# Autodesk Inventor assembly: Battery Basket
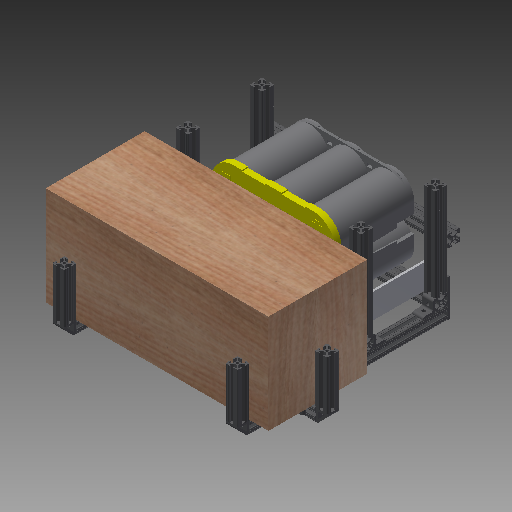
[picture p0: Inventor's stored thumbnail of the model, 512x512]
Saved by Autodesk Inventor 2017 SP1 (Build 210196100, 196)
## iProperties
Created: 2016-04-02
Part Number: Battery Basket
Document SubType Name: Assembly
Designer: hwasserb
Author: hwasserb
## Documents named in this file (14)
- C:\Users\Haden\Desktop\Charlie-CAD-Model\Robot Model\Battery Basket\Battery Basket.iam
- C:\Users\Haden\Desktop\Charlie-CAD-Model\Robot Model\Battery Basket\Back.ipt
- C:\Users\Haden\Desktop\Charlie-CAD-Model\Robot Model\Battery Basket\Bottom.ipt
- C:\Users\Haden\Desktop\Charlie-CAD-Model\Robot Model\Battery Basket\Right Angle.ipt
- C:\Users\Haden\Desktop\Charlie-CAD-Model\Robot Model\Battery Basket\Small Vertical.ipt
- C:\Users\Haden\Desktop\Charlie-CAD-Model\Robot Model\Battery Basket\Optima Battery.ipt
- C:\Users\Haden\Desktop\Charlie-CAD-Model\Robot Model\Battery Basket\Payload Lower Supports.ipt
- C:\Users\Haden\Desktop\Charlie-CAD-Model\Robot Model\Battery Basket\Inside Angle Connector-8020-4119.ipt
- C:\Users\Haden\Desktop\Charlie-CAD-Model\Robot Model\Battery Basket\3 Hole Plate-8020-4118.ipt
- C:\Users\Haden\Desktop\Charlie-CAD-Model\Robot Model\Payload.ipt
- C:\Users\Haden\Desktop\Charlie-CAD-Model\Robot Model\Battery Basket\1.5 Inch Spacer.ipt
- C:\Users\Haden\Desktop\Charlie-CAD-Model\Robot Model\Battery Basket\2 Hole Corner Bracket-8020-4132.ipt
- C:\Users\Haden\Desktop\Charlie-CAD-Model\Robot Model\Battery Basket\Payload Edge Guards.ipt
- C:\Users\Haden\Desktop\Charlie-CAD-Model\Robot Model\Battery Basket\1.75 Inch Spacer.ipt
## Components (39 placed, 13 different names)
1. Back:1 — Mate:23, Flush:3, Flush:4, Mate:64
2. Bottom:1 — Flush:1, Flush:2, Mate:1, Mate:2, Mate:3, Mate:4, Mate:5, Mate:6, Mate:32, Flush:8, Mate:36, Flush:10, Flush:11, Mate:39, Flush:12, Mate:40, Flush:13, Mate:65
3. Bottom:2 — Flush:1, Flush:2, Mate:7, Mate:8, Mate:9, Mate:10, Mate:27, Flush:5, Mate:28, Flush:6, Mate:29, Flush:7, Mate:34, Flush:9, Flush:14, Flush:15, Flush:16
4. Right Angle:1 — Mate:1, Mate:2, Mate:3, Mate:7, Mate:8, Mate:11, Mate:13, Mate:15, Mate:16, Mate:17, Mate:18
5. Right Angle:2 — Mate:4, Mate:5, Mate:6, Mate:9, Mate:10, Mate:12, Mate:14, Mate:19, Mate:20, Mate:21, Mate:22
6. Small Vertical:1 — Mate:13, Mate:15, Mate:16, Mate:26, Mate:47, Flush:27, Flush:28
7. Small Vertical:2 — Mate:14, Mate:19, Mate:20, Mate:45, Flush:21, Flush:22
8. Small Vertical:3 — Mate:12, Mate:21, Mate:22, Mate:44, Flush:23, Flush:24
9. Small Vertical:4 — Mate:11, Mate:17, Mate:18, Mate:23, Flush:3, Flush:4, Mate:46, Flush:25, Flush:26
10. Optima Battery:1 — Mate:26, Mate:64, Mate:65
11. Payload Lower Supports:1 — Mate:27, Flush:5, Mate:30, Mate:31, Mate:37, Flush:14, Mate:41, Flush:17, Insert:6, Flush:34, Flush:37, Mate:51, Mate:54, Flush:38, Mate:59, Flush:41
12. Payload Lower Supports:2 — Mate:28, Flush:6, Mate:33, Mate:35, Mate:38, Flush:13, Mate:42, Flush:18, Mate:43, Flush:19, Flush:20, Insert:5, Flush:35, Mate:50, Flush:36, Mate:57, Flush:39, Mate:58, Flush:40
13. Inside Angle Connector-8020-4119:1 — Mate:29, Flush:7, Mate:30
14. Inside Angle Connector-8020-4119:2 — Mate:33, Mate:34, Flush:9
15. Inside Angle Connector-8020-4119:3 — Mate:31, Mate:32, Flush:8
16. Inside Angle Connector-8020-4119:4 — Mate:35, Mate:36, Flush:10
17. Inside Angle Connector-8020-4119:5 — Mate:37, Flush:11, Mate:39
18. Inside Angle Connector-8020-4119:6 — Mate:38, Flush:12, Mate:40
19. 3 Hole Plate-8020-4118:1 — Mate:41, Flush:16, Flush:17
20. 3 Hole Plate-8020-4118:2 — Mate:42, Flush:15, Flush:18
21. Payload:1 — Mate:43, Flush:19, Flush:20, Flush:45
22. 1.5 Inch Spacer:3 — Mate:46, Flush:25, Flush:26
23. 1.5 Inch Spacer:4 — Mate:44, Flush:23, Flush:24
24. 1.5 Inch Spacer:5 — Mate:47, Flush:27, Flush:28
25. 1.5 Inch Spacer:6 — Mate:45, Flush:21, Flush:22
26. Payload Edge Guards:1 — Insert:4, Flush:43
27. Payload Edge Guards:2 — Insert:2, Flush:44
28. Payload Edge Guards:3 — Flush:34, Insert:7
29. Payload Edge Guards:4 — Flush:35, Insert:8
30. 2 Hole Corner Bracket-8020-4132:1 — Insert:2, Insert:10
31. 2 Hole Corner Bracket-8020-4132:2 — Insert:4, Insert:9
32. 2 Hole Corner Bracket-8020-4132:3 — Insert:5, Insert:8
33. 2 Hole Corner Bracket-8020-4132:4 — Insert:6, Insert:7
34. Inside Angle Connector-8020-4119:7 — Mate:57, Flush:39, Mate:60
35. Inside Angle Connector-8020-4119:8 — Mate:50, Flush:36, Mate:61
36. Inside Angle Connector-8020-4119:9 — Flush:37, Mate:51, Mate:63
37. Inside Angle Connector-8020-4119:10 — Mate:54, Flush:38, Mate:62
38. 1.75 Inch Spacer:1 — Mate:58, Flush:40, Flush:42, Mate:60, Mate:61, Insert:9, Flush:43, Flush:45
39. 1.75 Inch Spacer:2 — Mate:59, Flush:41, Flush:42, Mate:62, Mate:63, Insert:10, Flush:44
## Relationships (105: Mate 57, Flush 40, Insert 8)
- Flush:1: Bottom:1 ↔ Bottom:2
- Flush:2: Bottom:1 ↔ Bottom:2
- Mate:1: Bottom:1 ↔ Right Angle:1
- Mate:2: Bottom:1 ↔ Right Angle:1
- Mate:3: Bottom:1 ↔ Right Angle:1
- Mate:4: Bottom:1 ↔ Right Angle:2
- Mate:5: Bottom:1 ↔ Right Angle:2
- Mate:6: Bottom:1 ↔ Right Angle:2
- Mate:7: Bottom:2 ↔ Right Angle:1
- Mate:8: Bottom:2 ↔ Right Angle:1
- Mate:9: Bottom:2 ↔ Right Angle:2
- Mate:10: Bottom:2 ↔ Right Angle:2
- Mate:11: Right Angle:1 ↔ Small Vertical:4
- Mate:12: Right Angle:2 ↔ Small Vertical:3
- Mate:13: Right Angle:1 ↔ Small Vertical:1
- Mate:14: Right Angle:2 ↔ Small Vertical:2
- Mate:15: Right Angle:1 ↔ Small Vertical:1
- Mate:16: Right Angle:1 ↔ Small Vertical:1
- Mate:17: Right Angle:1 ↔ Small Vertical:4
- Mate:18: Right Angle:1 ↔ Small Vertical:4
- Mate:19: Right Angle:2 ↔ Small Vertical:2
- Mate:20: Right Angle:2 ↔ Small Vertical:2
- Mate:21: Right Angle:2 ↔ Small Vertical:3
- Mate:22: Right Angle:2 ↔ Small Vertical:3
- Mate:23: Back:1 ↔ Small Vertical:4
- Flush:3: Back:1 ↔ Small Vertical:4
- Flush:4 (-76.2 mm): Back:1 ↔ Small Vertical:4
- Mate:26 (38.1 mm): Small Vertical:1 ↔ Optima Battery:1
- Mate:27: Bottom:2 ↔ Payload Lower Supports:1
- Flush:5: Bottom:2 ↔ Payload Lower Supports:1
- Mate:28: Bottom:2 ↔ Payload Lower Supports:2
- Flush:6: Bottom:2 ↔ Payload Lower Supports:2
- Mate:29: Bottom:2 ↔ Inside Angle Connector-8020-4119:1
- Flush:7: Bottom:2 ↔ Inside Angle Connector-8020-4119:1
- Mate:30: Payload Lower Supports:1 ↔ Inside Angle Connector-8020-4119:1
- Mate:31: Payload Lower Supports:1 ↔ Inside Angle Connector-8020-4119:3
- Mate:32: Bottom:1 ↔ Inside Angle Connector-8020-4119:3
- Flush:8: Bottom:1 ↔ Inside Angle Connector-8020-4119:3
- Mate:33: Payload Lower Supports:2 ↔ Inside Angle Connector-8020-4119:2
- Mate:34: Bottom:2 ↔ Inside Angle Connector-8020-4119:2
- Flush:9: Bottom:2 ↔ Inside Angle Connector-8020-4119:2
- Mate:35: Payload Lower Supports:2 ↔ Inside Angle Connector-8020-4119:4
- Mate:36: Bottom:1 ↔ Inside Angle Connector-8020-4119:4
- Flush:10: Bottom:1 ↔ Inside Angle Connector-8020-4119:4
- Mate:37: Payload Lower Supports:1 ↔ Inside Angle Connector-8020-4119:5
- Mate:38: Payload Lower Supports:2 ↔ Inside Angle Connector-8020-4119:6
- Flush:11: Bottom:1 ↔ Inside Angle Connector-8020-4119:5
- Mate:39: Bottom:1 ↔ Inside Angle Connector-8020-4119:5
- Flush:12: Bottom:1 ↔ Inside Angle Connector-8020-4119:6
- Mate:40: Bottom:1 ↔ Inside Angle Connector-8020-4119:6
- Flush:13: Bottom:1 ↔ Payload Lower Supports:2
- Flush:14: Bottom:2 ↔ Payload Lower Supports:1
- Mate:41: Payload Lower Supports:1 ↔ 3 Hole Plate-8020-4118:1
- Mate:42: Payload Lower Supports:2 ↔ 3 Hole Plate-8020-4118:2
- Flush:15: Bottom:2 ↔ 3 Hole Plate-8020-4118:2
- Flush:16: Bottom:2 ↔ 3 Hole Plate-8020-4118:1
- Flush:17: Payload Lower Supports:1 ↔ 3 Hole Plate-8020-4118:1
- Flush:18: Payload Lower Supports:2 ↔ 3 Hole Plate-8020-4118:2
- Mate:43: Payload Lower Supports:2 ↔ Payload:1
- Flush:19: Payload Lower Supports:2 ↔ Payload:1
- Flush:20 (-38.1 mm): Payload Lower Supports:2 ↔ Payload:1
- Mate:44: Small Vertical:3 ↔ 1.5 Inch Spacer:4
- Mate:45: Small Vertical:2 ↔ 1.5 Inch Spacer:6
- Mate:46: Small Vertical:4 ↔ 1.5 Inch Spacer:3
- Mate:47: Small Vertical:1 ↔ 1.5 Inch Spacer:5
- Flush:21: Small Vertical:2 ↔ 1.5 Inch Spacer:6
- Flush:22: Small Vertical:2 ↔ 1.5 Inch Spacer:6
- Flush:23: Small Vertical:3 ↔ 1.5 Inch Spacer:4
- Flush:24: Small Vertical:3 ↔ 1.5 Inch Spacer:4
- Flush:25: Small Vertical:4 ↔ 1.5 Inch Spacer:3
- Flush:26: Small Vertical:4 ↔ 1.5 Inch Spacer:3
- Flush:27: Small Vertical:1 ↔ 1.5 Inch Spacer:5
- Flush:28: Small Vertical:1 ↔ 1.5 Inch Spacer:5
- Insert:2: Payload Edge Guards:2 ↔ 2 Hole Corner Bracket-8020-4132:1
- Insert:4: Payload Edge Guards:1 ↔ 2 Hole Corner Bracket-8020-4132:2
- Insert:5: Payload Lower Supports:2 ↔ 2 Hole Corner Bracket-8020-4132:3
- Insert:6: Payload Lower Supports:1 ↔ 2 Hole Corner Bracket-8020-4132:4
- Flush:34: Payload Lower Supports:1 ↔ Payload Edge Guards:3
- Flush:35: Payload Lower Supports:2 ↔ Payload Edge Guards:4
- Insert:7: Payload Edge Guards:3 ↔ 2 Hole Corner Bracket-8020-4132:4
- Insert:8: Payload Edge Guards:4 ↔ 2 Hole Corner Bracket-8020-4132:3
- Mate:50: Payload Lower Supports:2 ↔ Inside Angle Connector-8020-4119:8
- Flush:36: Payload Lower Supports:2 ↔ Inside Angle Connector-8020-4119:8
- Flush:37: Payload Lower Supports:1 ↔ Inside Angle Connector-8020-4119:9
- Mate:51: Payload Lower Supports:1 ↔ Inside Angle Connector-8020-4119:9
- Mate:54: Payload Lower Supports:1 ↔ Inside Angle Connector-8020-4119:10
- Flush:38: Payload Lower Supports:1 ↔ Inside Angle Connector-8020-4119:10
- Mate:57: Payload Lower Supports:2 ↔ Inside Angle Connector-8020-4119:7
- Flush:39: Payload Lower Supports:2 ↔ Inside Angle Connector-8020-4119:7
- Mate:58: Payload Lower Supports:2 ↔ 1.75 Inch Spacer:1
- Flush:40: Payload Lower Supports:2 ↔ 1.75 Inch Spacer:1
- Mate:59: Payload Lower Supports:1 ↔ 1.75 Inch Spacer:2
- Flush:41: Payload Lower Supports:1 ↔ 1.75 Inch Spacer:2
- Flush:42: 1.75 Inch Spacer:1 ↔ 1.75 Inch Spacer:2
- Mate:60: Inside Angle Connector-8020-4119:7 ↔ 1.75 Inch Spacer:1
- Mate:61: Inside Angle Connector-8020-4119:8 ↔ 1.75 Inch Spacer:1
- Mate:62: Inside Angle Connector-8020-4119:10 ↔ 1.75 Inch Spacer:2
- Mate:63: Inside Angle Connector-8020-4119:9 ↔ 1.75 Inch Spacer:2
- Insert:9: 2 Hole Corner Bracket-8020-4132:2 ↔ 1.75 Inch Spacer:1
- Insert:10: 2 Hole Corner Bracket-8020-4132:1 ↔ 1.75 Inch Spacer:2
- Flush:43: Payload Edge Guards:1 ↔ 1.75 Inch Spacer:1
- Flush:44: Payload Edge Guards:2 ↔ 1.75 Inch Spacer:2
- Flush:45 (88.9 mm): Payload:1 ↔ 1.75 Inch Spacer:1
- Mate:64: Back:1 ↔ Optima Battery:1
- Mate:65: Bottom:1 ↔ Optima Battery:1
